# Autodesk Inventor assembly: ARM
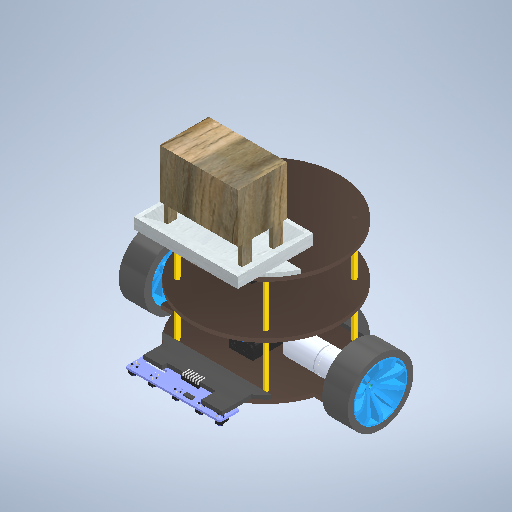
[picture p0: Inventor's stored thumbnail of the model, 512x512]
Saved by Autodesk Inventor 2025.2 (Build 292293000, 293)
## iProperties
Created: 2025-11-06
Part Number: ARM
Document SubType Name: Assembly
Designer: Dax
Author: Dax
## Documents named in this file (17)
- C:\Users\Dax\Documents\Tesis\MODELADO CAD\ARM\ARM.iam
- C:\Users\Dax\Documents\Tesis\MODELADO CAD\ARM\Base_inferior.ipt
- C:\Users\Dax\Documents\Tesis\MODELADO CAD\ARM\Soportes.ipt
- C:\Users\Dax\Documents\Tesis\MODELADO CAD\ARM\dc-motor-with-encoder-1.snapshot.1\Motor\Motor\Motor.ipt
- C:\Users\Dax\Documents\Tesis\MODELADO CAD\ARM\battery-holder-2-x-aaa.snapshot.2\battery holder 2 x AAA\battery holder 2 x AAA\battery holder 2 x AAA.ipt
- C:\Users\Dax\Documents\Tesis\MODELADO CAD\ARM\caster-ball-wheel-2.snapshot.1\caster ball wheel\caster ball wheel\caster ball wheel.ipt
- C:\Users\Dax\Documents\Tesis\MODELADO CAD\ARM\acople-eje-motor-de-3-o-4mm-1.snapshot.1\Coupling_4mmShaft\Coupling_4mmShaft\Coupling_4mmShaft.ipt
- C:\Users\Dax\Documents\Tesis\MODELADO CAD\ARM\model-rc-wheel-1.snapshot.1\Tires\Tires\Tires.ipt
- C:\Users\Dax\Documents\Tesis\MODELADO CAD\ARM\follower sensor\TCRT5000 v1.iam
- C:\Users\Dax\Documents\Tesis\MODELADO CAD\ARM\Plataforma.ipt
- C:\Users\Dax\Documents\Tesis\MODELADO CAD\ARM\esp32-devkit_1-shield-expansion-board-1.snapshot.10\Shield ESP32\Shield ESP32\Shield ESP32.ipt
- C:\Users\Dax\Documents\Tesis\MODELADO CAD\ARM\dc-dc-lm2596-3a-step-down-converter-module-1.snapshot.5\HW-411\HW-411\HW-411.ipt
- C:\Users\Dax\Documents\Tesis\MODELADO CAD\ARM\motor-driver-4.snapshot.1\Motor Driver\Motor Driver\Motor Driver.ipt
- C:\Users\Dax\Documents\Tesis\MODELADO CAD\ARM\Viga.ipt
- C:\Users\Dax\Documents\Tesis\MODELADO CAD\ARM\nvidia-jetson-nano-3.snapshot.1\22-5-12 NVIDIA jetson nano\jetson nano\jetson nano\jetson nano.ipt
- C:\Users\Dax\Documents\Tesis\MODELADO CAD\ARM\Soporte_caja.ipt
- C:\Users\Dax\Documents\Tesis\MODELADO CAD\ARM\Caja.ipt
## Components (28 placed, 16 different names)
1. Base_inferior:1 — Coincidencia:1, Coincidencia:2, Coincidencia:3, Coincidencia:4, Coincidencia:5, Nivelación:1, Tangente:1, Coincidencia:6, Nivelación:2, Tangente:2, Nivelación:3, Coincidencia:7, Coincidencia:8, Coincidencia:9, Tangente:3, Coincidencia:11, Tangente:4, Coincidencia:13, Coincidencia:25, Coincidencia:26, Coincidencia:27, Coincidencia:30, Coincidencia:37, Coincidencia:38, Coincidencia:39, Coincidencia:40, Coincidencia:41, Coincidencia:42, Coincidencia:43, Coincidencia:44
2. Soportes:2 — Coincidencia:4, Coincidencia:5, Coincidencia:10, Coincidencia:12, Coincidencia:27, Coincidencia:28, Coincidencia:29
3. Motor:1 — Nivelación:1, Tangente:1, Coincidencia:6, Coincidencia:15, Coincidencia:17
4. Motor:3 — Nivelación:2, Tangente:2, Nivelación:3, Coincidencia:14, Coincidencia:16
5. battery holder 2 x AAA:1 — Coincidencia:7, Coincidencia:8, Coincidencia:9
6. caster ball wheel:1 — Coincidencia:10, Tangente:3, Coincidencia:11
7. caster ball wheel:2 — Coincidencia:12, Tangente:4, Coincidencia:13
8. Coupling_4mmShaft:1 — Coincidencia:15, Coincidencia:17, Coincidencia:20, Coincidencia:22, Coincidencia:24
9. Coupling_4mmShaft:2 — Coincidencia:14, Coincidencia:16, Coincidencia:19, Coincidencia:21, Coincidencia:23
10. Tires:1 — Coincidencia:21, Coincidencia:23, Coincidencia:25
11. Tires:2 — Coincidencia:22, Coincidencia:24, Coincidencia:26
12. TCRT5000 v1:5 [sub-assembly] — Coincidencia:28, Coincidencia:29, Coincidencia:30
13. Plataforma:1 — Coincidencia:31, Coincidencia:32, Tangente:5, Coincidencia:33, Coincidencia:34, Tangente:6, Coincidencia:35, Coincidencia:36, Tangente:7, Coincidencia:45, Coincidencia:46, Coincidencia:47, Coincidencia:48, Coincidencia:49, Coincidencia:50, Coincidencia:51, Coincidencia:52, Coincidencia:53, Coincidencia:54, Coincidencia:55
14. Shield ESP32:1 — Coincidencia:31, Coincidencia:32, Tangente:5
15. HW-411:1 — Coincidencia:35, Coincidencia:36, Tangente:7
16. Motor Driver:1 — Coincidencia:33, Coincidencia:34, Tangente:6
17. Viga:1 — Coincidencia:37, Coincidencia:38
18. Viga:2 — Coincidencia:39, Coincidencia:40, Coincidencia:55
19. Viga:3 — Coincidencia:41, Coincidencia:42, Coincidencia:45, Coincidencia:46
20. Viga:4 — Coincidencia:43, Coincidencia:44
21. Viga:5 — Coincidencia:47, Coincidencia:51, Coincidencia:60
22. Viga:6 — Coincidencia:50, Coincidencia:52, Coincidencia:59
23. Viga:7 — Coincidencia:48, Coincidencia:54
24. Viga:8 — Coincidencia:49, Coincidencia:53, Coincidencia:58
25. Plataforma:2 — Coincidencia:56, Coincidencia:57, Tangente:8, Coincidencia:58, Coincidencia:59, Coincidencia:60, Coincidencia:61, Coincidencia:62, Coincidencia:63
26. jetson nano:1 — Coincidencia:56, Coincidencia:57, Tangente:8
27. Soporte_caja:2 — Coincidencia:61, Coincidencia:62, Coincidencia:63, Coincidencia:64, Coincidencia:65, Coincidencia:66
28. Caja:1 — Coincidencia:64, Coincidencia:65, Coincidencia:66
## Relationships (76: Mate 65, Tangent 8, Flush 3)
- Coincidencia:1 [Mate]: Base_inferior:1
- Coincidencia:2 [Mate]: Base_inferior:1
- Coincidencia:3 [Mate]: Base_inferior:1
- Coincidencia:4 [Mate]: Base_inferior:1 ↔ Soportes:2
- Coincidencia:5 [Mate]: Base_inferior:1 ↔ Soportes:2
- Nivelación:1 [Flush]: Base_inferior:1 ↔ Motor:1
- Tangente:1: Base_inferior:1 ↔ Motor:1
- Coincidencia:6 [Mate]: Base_inferior:1 ↔ Motor:1
- Nivelación:2 [Flush]: Base_inferior:1 ↔ Motor:3
- Tangente:2: Base_inferior:1 ↔ Motor:3
- Nivelación:3 [Flush]: Base_inferior:1 ↔ Motor:3
- Coincidencia:7 [Mate]: Base_inferior:1 ↔ battery holder 2 x AAA:1
- Coincidencia:8 [Mate]: Base_inferior:1 ↔ battery holder 2 x AAA:1
- Coincidencia:9 [Mate]: Base_inferior:1 ↔ battery holder 2 x AAA:1
- Coincidencia:10 [Mate]: Soportes:2 ↔ caster ball wheel:1
- Tangente:3 (2 mm): Base_inferior:1 ↔ caster ball wheel:1
- Coincidencia:11 [Mate]: Base_inferior:1 ↔ caster ball wheel:1
- Coincidencia:12 [Mate]: Soportes:2 ↔ caster ball wheel:2
- Tangente:4 (2 mm): Base_inferior:1 ↔ caster ball wheel:2
- Coincidencia:13 [Mate]: Base_inferior:1 ↔ caster ball wheel:2
- Coincidencia:14 [Mate]: Motor:3 ↔ Coupling_4mmShaft:2
- Coincidencia:15 [Mate]: Motor:1 ↔ Coupling_4mmShaft:1
- Coincidencia:16 [Mate]: Motor:3 ↔ Coupling_4mmShaft:2
- Coincidencia:17 [Mate]: Motor:1 ↔ Coupling_4mmShaft:1
- Coincidencia:19 [Mate]: Coupling_4mmShaft:2
- Coincidencia:20 [Mate]: Coupling_4mmShaft:1
- Coincidencia:21 [Mate]: Coupling_4mmShaft:2 ↔ Tires:1
- Coincidencia:22 [Mate]: Coupling_4mmShaft:1 ↔ Tires:2
- Coincidencia:23 [Mate]: Coupling_4mmShaft:2 ↔ Tires:1
- Coincidencia:24 [Mate]: Coupling_4mmShaft:1 ↔ Tires:2
- Coincidencia:25 [Mate]: Base_inferior:1 ↔ Tires:1
- Coincidencia:26 [Mate]: Base_inferior:1 ↔ Tires:2
- Coincidencia:27 [Mate]: Base_inferior:1 ↔ Soportes:2
- Coincidencia:28 [Mate]: Soportes:2 ↔ TCRT5000 v1:5
- Coincidencia:29 [Mate]: Soportes:2 ↔ TCRT5000 v1:5
- Coincidencia:30 [Mate]: Base_inferior:1 ↔ TCRT5000 v1:5
- Coincidencia:31 [Mate]: Plataforma:1 ↔ Shield ESP32:1
- Coincidencia:32 [Mate]: Plataforma:1 ↔ Shield ESP32:1
- Tangente:5 (-8 mm): Plataforma:1 ↔ Shield ESP32:1
- Coincidencia:33 [Mate]: Plataforma:1 ↔ Motor Driver:1
- Coincidencia:34 [Mate] (15 mm): Plataforma:1 ↔ Motor Driver:1
- Tangente:6 (-20 mm): Plataforma:1 ↔ Motor Driver:1
- Coincidencia:35 [Mate]: Plataforma:1 ↔ HW-411:1
- Coincidencia:36 [Mate] (-15 mm): Plataforma:1 ↔ HW-411:1
- Tangente:7 (-20 mm): Plataforma:1 ↔ HW-411:1
- Coincidencia:37 [Mate]: Base_inferior:1 ↔ Viga:1
- Coincidencia:38 [Mate]: Base_inferior:1 ↔ Viga:1
- Coincidencia:39 [Mate]: Base_inferior:1 ↔ Viga:2
- Coincidencia:40 [Mate]: Base_inferior:1 ↔ Viga:2
- Coincidencia:41 [Mate]: Base_inferior:1 ↔ Viga:3
- Coincidencia:42 [Mate]: Base_inferior:1 ↔ Viga:3
- Coincidencia:43 [Mate]: Base_inferior:1 ↔ Viga:4
- Coincidencia:44 [Mate]: Base_inferior:1 ↔ Viga:4
- Coincidencia:45 [Mate]: Plataforma:1 ↔ Viga:3
- Coincidencia:46 [Mate]: Plataforma:1 ↔ Viga:3
- Coincidencia:47 [Mate]: Plataforma:1 ↔ Viga:5
- Coincidencia:48 [Mate]: Plataforma:1 ↔ Viga:7
- Coincidencia:49 [Mate]: Plataforma:1 ↔ Viga:8
- Coincidencia:50 [Mate]: Plataforma:1 ↔ Viga:6
- Coincidencia:51 [Mate]: Plataforma:1 ↔ Viga:5
- Coincidencia:52 [Mate]: Plataforma:1 ↔ Viga:6
- Coincidencia:53 [Mate]: Plataforma:1 ↔ Viga:8
- Coincidencia:54 [Mate]: Plataforma:1 ↔ Viga:7
- Coincidencia:55 [Mate]: Plataforma:1 ↔ Viga:2
- Coincidencia:56 [Mate]: Plataforma:2 ↔ jetson nano:1
- Coincidencia:57 [Mate]: Plataforma:2 ↔ jetson nano:1
- Tangente:8 (-40 mm): Plataforma:2 ↔ jetson nano:1
- Coincidencia:58 [Mate]: Viga:8 ↔ Plataforma:2
- Coincidencia:59 [Mate]: Viga:6 ↔ Plataforma:2
- Coincidencia:60 [Mate]: Viga:5 ↔ Plataforma:2
- Coincidencia:61 [Mate]: Plataforma:2 ↔ Soporte_caja:2
- Coincidencia:62 [Mate]: Plataforma:2 ↔ Soporte_caja:2
- Coincidencia:63 [Mate]: Plataforma:2 ↔ Soporte_caja:2
- Coincidencia:64 [Mate]: Soporte_caja:2 ↔ Caja:1
- Coincidencia:65 [Mate]: Soporte_caja:2 ↔ Caja:1
- Coincidencia:66 [Mate]: Soporte_caja:2 ↔ Caja:1
